# Autodesk Inventor assembly: circuito montado
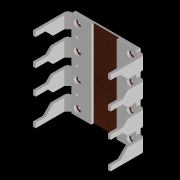
[picture p0: Inventor's stored thumbnail of the model, 180x180]
Saved by Autodesk Inventor 2020 (Build 240168000, 168)
## iProperties
Created: 2020-02-11
Part Number: circuito montado
Document SubType Name: Assembly
Designer: PEDRO
Author: PEDRO
## Documents named in this file (4)
- C:\Users\PEDRO\Desktop\555 Transistores\circuito montado.iam
- C:\Users\PEDRO\Desktop\555 Transistores\suporte 555 parte 1.ipt
- C:\Users\PEDRO\Desktop\555 Transistores\suporte 555 parte 2.ipt
- C:\Users\PEDRO\Desktop\555 Transistores\Placa.ipt
## Components (3 placed, 3 different names)
1. suporte 555 parte 1:1 — Flush:1, Flush:2, Mate:1, Mate:2
2. suporte 555 parte 2:1 — Flush:1, Flush:2, Mate:3, Mate:4, Mate:5
3. Placa:1 — Mate:1, Mate:2, Mate:3, Mate:4, Mate:5
## Relationships (7: Mate 5, Flush 2)
- Flush:1: suporte 555 parte 1:1 ↔ suporte 555 parte 2:1
- Flush:2: suporte 555 parte 1:1 ↔ suporte 555 parte 2:1
- Mate:1: suporte 555 parte 1:1 ↔ Placa:1
- Mate:2: suporte 555 parte 1:1 ↔ Placa:1
- Mate:3: suporte 555 parte 2:1 ↔ Placa:1
- Mate:4: suporte 555 parte 2:1 ↔ Placa:1
- Mate:5: suporte 555 parte 2:1 ↔ Placa:1
